# Autodesk Inventor assembly: Robot Frame
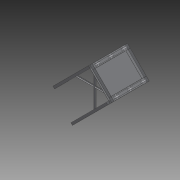
[picture p0: Inventor's stored thumbnail of the model, 180x180]
Saved by Autodesk Inventor 2015 (Build 190159000, 159)
## iProperties
Created: 2015-01-10
Part Number: Robot Frame
Document SubType Name: Assembly
Designer: Chandler Willoughby
Author: Chandler Willoughby
## Documents named in this file (12)
- C:\Autodesk\FIRST\Simple Parts\Robot Frame.iam
- C:\Autodesk\FIRST\Simple Parts\Frame.ipt
- C:\Autodesk\FIRST\Simple Parts\L-Frame.ipt
- C:\Autodesk\FIRST\Simple Parts\Front Right Beam.ipt
- C:\Autodesk\FIRST\Simple Parts\Front Left Beam.ipt
- C:\Autodesk\FIRST\Simple Parts\L-Frame Small.ipt
- C:\Autodesk\FIRST\Simple Parts\Base.ipt
- C:\Autodesk\FIRST\Simple Parts\Wheel.ipt
- C:\Autodesk\FIRST\Simple Parts\Brace Back Horizontal.ipt
- C:\Autodesk\FIRST\Simple Parts\Brace Back 45.ipt
- C:\Autodesk\FIRST\Simple Parts\Brace Back 45 B.ipt
- C:\Autodesk\FIRST\Simple Parts\Top Frame Left.ipt
## Components (22 placed, 11 different names)
1. Frame:1 — Mate:1, Flush:1, Flush:2, Mate:2, Flush:3, Flush:4, Mate:4, Flush:7, Angle:1, Mate:5, Flush:9, Mate:6, Mate:7, Mate:8, Mate:9, Flush:10, Flush:11, Flush:12, Flush:13, Flush:14, Flush:15, Flush:16, Flush:17
2. L-Frame:1 — Mate:1, Flush:1, Flush:2, Mate:12, Mate:13, Mate:14, Mate:15, Mate:16, Mate:19, Mate:20, Mate:21, Mate:22, Mate:23, Mate:24, Mate:25, Mate:26, Flush:21
3. L-Frame:2 — Mate:2, Flush:3, Flush:4
4. Front Right Beam:1 — Mate:4, Flush:7, Angle:1
5. Front Left Beam:1 — Mate:5, Flush:9, Flush:20
6. L-Frame Small:1 — Mate:9, Flush:10, Flush:11, Mate:11
7. L-Frame Small:2 — Mate:8, Flush:14, Flush:15, Mate:10
8. L-Frame Small:3 — Mate:6, Flush:12, Flush:13
9. L-Frame Small:4 — Mate:7, Flush:16, Flush:17, Flush:18, Flush:19
10. Base:1 — Mate:10, Mate:11, Flush:18, Flush:19, Insert:1, Insert:2, Insert:3, Insert:4, Insert:5, Insert:6
11. Wheel:1 — Insert:1
12. Wheel:2 — Insert:2
13. Wheel:3 — Insert:5
14. Wheel:4 — Insert:3
15. Wheel:5 — Insert:4
16. Wheel:6 — Insert:6
17. Brace Back Horizontal:1 — Mate:12, Mate:13
18. Brace Back 45:1 — Mate:14, Mate:16, Mate:19
19. Brace Back 45:2 — Mate:15, Mate:20
20. Brace Back 45 B:1 — Mate:22, Mate:24
21. Brace Back 45 B:2 — Mate:21, Mate:23
22. Top Frame Left:1 — Mate:25, Mate:26, Flush:20, Flush:21
## Relationships (48: Mate 23, Flush 18, Insert 6, Angle 1)
- Mate:1: Frame:1 ↔ L-Frame:1
- Flush:1: Frame:1 ↔ L-Frame:1
- Flush:2: Frame:1 ↔ L-Frame:1
- Mate:2: Frame:1 ↔ L-Frame:2
- Flush:3: Frame:1 ↔ L-Frame:2
- Flush:4: Frame:1 ↔ L-Frame:2
- Mate:4: Frame:1 ↔ Front Right Beam:1
- Flush:7: Frame:1 ↔ Front Right Beam:1
- Angle:1 (14.78 deg): Frame:1 ↔ Front Right Beam:1
- Mate:5: Frame:1 ↔ Front Left Beam:1
- Flush:9: Frame:1 ↔ Front Left Beam:1
- Mate:6: Frame:1 ↔ L-Frame Small:3
- Mate:7: Frame:1 ↔ L-Frame Small:4
- Mate:8: Frame:1 ↔ L-Frame Small:2
- Mate:9: Frame:1 ↔ L-Frame Small:1
- Flush:10: Frame:1 ↔ L-Frame Small:1
- Flush:11: Frame:1 ↔ L-Frame Small:1
- Flush:12: Frame:1 ↔ L-Frame Small:3
- Flush:13: Frame:1 ↔ L-Frame Small:3
- Flush:14: Frame:1 ↔ L-Frame Small:2
- Flush:15: Frame:1 ↔ L-Frame Small:2
- Flush:16: Frame:1 ↔ L-Frame Small:4
- Flush:17: Frame:1 ↔ L-Frame Small:4
- Mate:10: L-Frame Small:2 ↔ Base:1
- Mate:11: L-Frame Small:1 ↔ Base:1
- Flush:18: L-Frame Small:4 ↔ Base:1
- Flush:19: L-Frame Small:4 ↔ Base:1
- Insert:1: Base:1 ↔ Wheel:1
- Insert:2: Base:1 ↔ Wheel:2
- Insert:3: Base:1 ↔ Wheel:4
- Insert:4: Base:1 ↔ Wheel:5
- Insert:5: Base:1 ↔ Wheel:3
- Insert:6: Base:1 ↔ Wheel:6
- Mate:12: L-Frame:1 ↔ Brace Back Horizontal:1
- Mate:13: L-Frame:1 ↔ Brace Back Horizontal:1
- Mate:14: L-Frame:1 ↔ Brace Back 45:1
- Mate:15: L-Frame:1 ↔ Brace Back 45:2
- Mate:16: L-Frame:1 ↔ Brace Back 45:1
- Mate:19: L-Frame:1 ↔ Brace Back 45:1
- Mate:20: L-Frame:1 ↔ Brace Back 45:2
- Mate:21: L-Frame:1 ↔ Brace Back 45 B:2
- Mate:22: L-Frame:1 ↔ Brace Back 45 B:1
- Mate:23: L-Frame:1 ↔ Brace Back 45 B:2
- Mate:24: L-Frame:1 ↔ Brace Back 45 B:1
- Mate:25: L-Frame:1 ↔ Top Frame Left:1
- Mate:26: L-Frame:1 ↔ Top Frame Left:1
- Flush:20: Front Left Beam:1 ↔ Top Frame Left:1
- Flush:21: L-Frame:1 ↔ Top Frame Left:1
